# Autodesk Inventor assembly: J005190
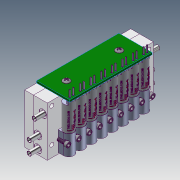
[picture p0: Inventor's stored thumbnail of the model, 180x180]
Saved by Autodesk Inventor 2015 SP1 (Build 190203100, 203)
## iProperties
RuleStatus: InUse
AfterDocSave0: file://Part Number Cleaner
Created: 2015-04-08
Vendor: HHMI: JRC - ID&F
Document SubType Name: Assembly
Designer: JORDANJ
Part Number: J005190
Description: COMPONENT OF AN AUTOMATED LIQUID HANDLING MACHINE SPECIFICALLY DESIGNED FOR THE IN SITU RNA HYBRIDIZATION OF DROSOPHILA EMBRYOS
Project: P-171601
DESIGN DEPARTMENT: HHMI: JRC - ID&F
LAB/DEPT: STERN (LAB)
REQUESTING SCIENTIST: STERN, DAVID
SPECIAL FINISH: NONE
SURFACE ROUGHNESS: N/A
ALTERED ITEM PART NUMBER: N/A
ALTERED ITEM VENDOR: N/A
ALTERED ITEM DESCRIPTION: N/A
Revision Number: 0
## Documents named in this file (13)
- C:\_WORKSPACE\DATA\PROJECTS\_PROJECTS BY LAB\STERN (LAB)\HYBRIDIZER\MCAD\MICROPLATE\24W CHEMICAL MANIFOLD.iam
- C:\_WORKSPACE\DATA\PROJECTS\_PROJECTS BY LAB\STERN (LAB)\HYBRIDIZER\MCAD\MICROPLATE\24W CHEM MANIFOLD 8X BASE.ipt
- C:\_WORKSPACE\DATA\PROJECTS\_PROJECTS BY LAB\STERN (LAB)\HYBRIDIZER\MCAD\MICROPLATE\24W CHEM MANIFOLD 8X COVER.ipt
- C:\_WORKSPACE\DATA\PROJECTS\_PROJECTS BY LAB\STERN (LAB)\HYBRIDIZER\MCAD\MICROPLATE\24W CHEM MANIFOLD PORT.ipt
- C:\_WORKSPACE\DATA\PROJECTS\_PROJECTS BY LAB\STERN (LAB)\HYBRIDIZER\MCAD\MICROPLATE\24W DUCKBILL VALVE 3.9.ipt
- C:\_WORKSPACE\DATA\PROJECTS\_PROJECTS BY LAB\STERN (LAB)\HYBRIDIZER\MCAD\MICROPLATE\_24W CHEMICAL MANIFOLD.ipt
- C:\_WORKSPACE\DATA\Imported Components\92196A079\92196A079.ipt
- C:\_WORKSPACE\DATA\PROJECTS\_PROJECTS BY LAB\STERN (LAB)\HYBRIDIZER\MCAD\MICROPLATE\24W CHEM MANIFOLD ORING.ipt
- C:\_WORKSPACE\DATA\Imported Components\LHDA FACEMOUNT GENERIC\LHDA FACEMOUNT EXTENDED PERFORMANCE GENERIC.ipt
- C:\_WORKSPACE\DATA\Imported Components\91771A242\91771A242.ipt
- C:\_WORKSPACE\DATA\Imported Components\91770A071\91770A071.ipt
- C:\_WORKSPACE\DATA\PROJECTS\_PROJECTS BY LAB\STERN (LAB)\HYBRIDIZER\MCAD\MICROPLATE\24W CHEMICAL SELECTION BOARD.ipt
- C:\_WORKSPACE\DATA\Imported Components\mill-max-0305-0-15-01-47-XX-10-0\mill-max-0305-0-15-01-47-XX-10-0.ipt
## Components (79 placed, 11 different names)
1. 24W CHEMICAL SELECTION BOARD:1 — Insert:10, Insert:11, Flush:10, Flush:11, Flush:12, Insert:15, Insert:16
2. 24W CHEM MANIFOLD 8X COVER:1 — Flush:4, Flush:5, Flush:6, Insert:2, Insert:3, Insert:12, Insert:13, Insert:14
3. 24W CHEM MANIFOLD 8X BASE:1 — Flush:1, Flush:2, Flush:3, Insert:1, Insert:4, Insert:5, Insert:6, Insert:7, Mate:1, Mate:2, Mate:3, Insert:17, Insert:18
4. 24W CHEM MANIFOLD PORT:18 — Insert:6
5. 24W CHEM MANIFOLD PORT:17 — Insert:7
6. 24W CHEM MANIFOLD PORT:19 — Insert:4
7. 24W CHEM MANIFOLD PORT:20 — Insert:5
8. 92196A079:2 — Insert:9
9. 91771A242:1 — Insert:12
10. 91771A242:2 — Insert:13
11. 91771A242:3 — Insert:14
12. 91770A071:1 — Insert:15
13. 91770A071:2 — Insert:16
14. 24W CHEM MANIFOLD PORT:21 — Insert:17
15. 24W CHEM MANIFOLD PORT:22 — Insert:18
16. 24W CHEM MANIFOLD PORT:2 — Insert:3
17. 24W CHEM MANIFOLD PORT:1 — Insert:2
18. 24W DUCKBILL VALVE 3.9:1 — Insert:1
19. LHDA FACEMOUNT EXTENDED PERFORMANCE GENERIC:1 — Mate:1, Mate:2, Mate:3, Insert:8
20. 92196A079:1 — Insert:8
21. 24W CHEM MANIFOLD ORING:1 — Flush:7, Flush:8, Flush:9
22. mill-max-0305-0-15-01-47-XX-10-0:1 — Insert:10
23. mill-max-0305-0-15-01-47-XX-10-0:2 — Insert:11
24. 24W CHEM MANIFOLD PORT:3
25. 24W CHEM MANIFOLD PORT:4
26. 24W DUCKBILL VALVE 3.9:2
27. LHDA FACEMOUNT EXTENDED PERFORMANCE GENERIC:2
28. 92196A079:3
29. 24W CHEM MANIFOLD ORING:2
30. mill-max-0305-0-15-01-47-XX-10-0:3
31. mill-max-0305-0-15-01-47-XX-10-0:10
32. 24W CHEM MANIFOLD PORT:5
33. 24W CHEM MANIFOLD PORT:6
34. 24W DUCKBILL VALVE 3.9:3
35. LHDA FACEMOUNT EXTENDED PERFORMANCE GENERIC:3
36. 92196A079:4
37. 24W CHEM MANIFOLD ORING:3
38. mill-max-0305-0-15-01-47-XX-10-0:4
39. mill-max-0305-0-15-01-47-XX-10-0:11
40. 24W CHEM MANIFOLD PORT:7
41. 24W CHEM MANIFOLD PORT:8
42. 24W DUCKBILL VALVE 3.9:4
43. LHDA FACEMOUNT EXTENDED PERFORMANCE GENERIC:4
44. 92196A079:5
45. 24W CHEM MANIFOLD ORING:4
46. mill-max-0305-0-15-01-47-XX-10-0:5
47. mill-max-0305-0-15-01-47-XX-10-0:12
48. 24W CHEM MANIFOLD PORT:9
49. 24W CHEM MANIFOLD PORT:10
50. 24W DUCKBILL VALVE 3.9:5
51. LHDA FACEMOUNT EXTENDED PERFORMANCE GENERIC:5
52. 92196A079:6
53. 24W CHEM MANIFOLD ORING:5
54. mill-max-0305-0-15-01-47-XX-10-0:6
55. mill-max-0305-0-15-01-47-XX-10-0:13
56. 24W CHEM MANIFOLD PORT:11
57. 24W CHEM MANIFOLD PORT:12
58. 24W DUCKBILL VALVE 3.9:6
59. LHDA FACEMOUNT EXTENDED PERFORMANCE GENERIC:6
60. 92196A079:7
61. 24W CHEM MANIFOLD ORING:6
62. mill-max-0305-0-15-01-47-XX-10-0:7
63. mill-max-0305-0-15-01-47-XX-10-0:14
64. 24W CHEM MANIFOLD PORT:13
65. 24W CHEM MANIFOLD PORT:14
66. 24W DUCKBILL VALVE 3.9:7
67. LHDA FACEMOUNT EXTENDED PERFORMANCE GENERIC:7
68. 92196A079:8
69. 24W CHEM MANIFOLD ORING:7
70. mill-max-0305-0-15-01-47-XX-10-0:8
71. mill-max-0305-0-15-01-47-XX-10-0:15
72. 24W CHEM MANIFOLD PORT:15
73. 24W CHEM MANIFOLD PORT:16
74. 24W DUCKBILL VALVE 3.9:8
75. LHDA FACEMOUNT EXTENDED PERFORMANCE GENERIC:8 — Insert:9
76. 92196A079:9
77. 24W CHEM MANIFOLD ORING:8
78. mill-max-0305-0-15-01-47-XX-10-0:9
79. mill-max-0305-0-15-01-47-XX-10-0:16
## Component patterns: (8 elements, first: 24W CHEM MANIFOLD PORT:2 + 24W CHEM MANIFOLD PORT:1 + 24W DUCKBILL VALVE 3.9:1 + LHDA FACEMOUNT EXTENDED PERFORMANCE GENERIC:1 + 92196A079:1 + 24W CHEM MANIFOLD ORING:1 + mill-max-0305-0-15-01-47-XX-10-0:1 + mill-max-0305-0-15-01-47-XX-10-0:2)
## Relationships (33: Insert 18, Flush 12, Mate 3)
- Flush:1: 24W CHEM MANIFOLD 8X BASE:1
- Flush:2: 24W CHEM MANIFOLD 8X BASE:1
- Flush:3: 24W CHEM MANIFOLD 8X BASE:1
- Flush:4: 24W CHEM MANIFOLD 8X COVER:1
- Flush:5: 24W CHEM MANIFOLD 8X COVER:1
- Flush:6: 24W CHEM MANIFOLD 8X COVER:1
- Insert:1: 24W CHEM MANIFOLD 8X BASE:1 ↔ 24W DUCKBILL VALVE 3.9:1
- Insert:2: 24W CHEM MANIFOLD 8X COVER:1 ↔ 24W CHEM MANIFOLD PORT:1
- Insert:3: 24W CHEM MANIFOLD 8X COVER:1 ↔ 24W CHEM MANIFOLD PORT:2
- Insert:4: 24W CHEM MANIFOLD 8X BASE:1 ↔ 24W CHEM MANIFOLD PORT:19
- Insert:5: 24W CHEM MANIFOLD 8X BASE:1 ↔ 24W CHEM MANIFOLD PORT:20
- Insert:6: 24W CHEM MANIFOLD 8X BASE:1 ↔ 24W CHEM MANIFOLD PORT:18
- Insert:7: 24W CHEM MANIFOLD 8X BASE:1 ↔ 24W CHEM MANIFOLD PORT:17
- Mate:1: 24W CHEM MANIFOLD 8X BASE:1 ↔ LHDA FACEMOUNT EXTENDED PERFORMANCE GENERIC:1
- Mate:2: 24W CHEM MANIFOLD 8X BASE:1 ↔ LHDA FACEMOUNT EXTENDED PERFORMANCE GENERIC:1
- Mate:3: 24W CHEM MANIFOLD 8X BASE:1 ↔ LHDA FACEMOUNT EXTENDED PERFORMANCE GENERIC:1
- Insert:8: LHDA FACEMOUNT EXTENDED PERFORMANCE GENERIC:1 ↔ 92196A079:1
- Insert:9: 92196A079:2 ↔ LHDA FACEMOUNT EXTENDED PERFORMANCE GENERIC:8
- Flush:7: 24W CHEM MANIFOLD ORING:1
- Flush:8: 24W CHEM MANIFOLD ORING:1
- Flush:9: 24W CHEM MANIFOLD ORING:1
- Insert:10: 24W CHEMICAL SELECTION BOARD:1 ↔ mill-max-0305-0-15-01-47-XX-10-0:1
- Insert:11: 24W CHEMICAL SELECTION BOARD:1 ↔ mill-max-0305-0-15-01-47-XX-10-0:2
- Flush:10: 24W CHEMICAL SELECTION BOARD:1
- Flush:11: 24W CHEMICAL SELECTION BOARD:1
- Flush:12: 24W CHEMICAL SELECTION BOARD:1
- Insert:12: 24W CHEM MANIFOLD 8X COVER:1 ↔ 91771A242:1
- Insert:13: 24W CHEM MANIFOLD 8X COVER:1 ↔ 91771A242:2
- Insert:14: 24W CHEM MANIFOLD 8X COVER:1 ↔ 91771A242:3
- Insert:15: 24W CHEMICAL SELECTION BOARD:1 ↔ 91770A071:1
- Insert:16: 24W CHEMICAL SELECTION BOARD:1 ↔ 91770A071:2
- Insert:17: 24W CHEM MANIFOLD 8X BASE:1 ↔ 24W CHEM MANIFOLD PORT:21
- Insert:18: 24W CHEM MANIFOLD 8X BASE:1 ↔ 24W CHEM MANIFOLD PORT:22
## Named parameters: valve_spacing = 7.62 mm, no_valves = 8
